# Autodesk Inventor assembly: LeftSideEBoard
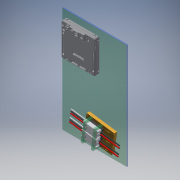
[picture p0: Inventor's stored thumbnail of the model, 180x180]
Saved by Autodesk Inventor 2019 (Build 230136000, 136)
## iProperties
Created: 2020-01-24
Part Number: LeftSideEBoard
Document SubType Name: Assembly
Designer: james
Author: james
## Documents named in this file (4)
- F:\JimsRobot\FIRSTRobots\Design\JimsCHS2020FRC\LeftSideEBoard.iam
- F:\JimsRobot\FIRSTRobots\Design\JimsCHS2020FRC\SideEBoard.ipt
- F:\JimsRobot\FIRSTRobots\Design\Library\AndyMark\roboRIO CAD\3d\cd_roborio.ipt
- F:\JimsRobot\FIRSTRobots\Design\Library\Jims\TwoSparkMaxPlate.iam
## Components (3 placed, 3 different names)
1. SideEBoard:1 — Mate:1, Mate:2
2. cd_roborio:1 — Mate:1
3. TwoSparkMaxPlate:1 [sub-assembly] — Mate:2
## Relationships (2: Mate 2)
- Mate:1: SideEBoard:1 ↔ cd_roborio:1
- Mate:2: SideEBoard:1 ↔ TwoSparkMaxPlate:1
